# Autodesk Inventor assembly: Butterfly Drive Module_MIR1
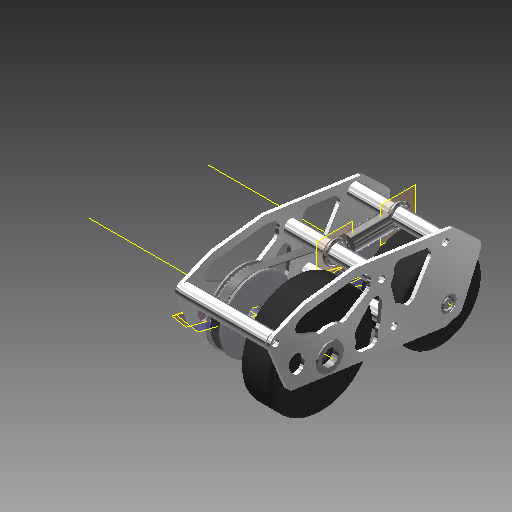
[picture p0: Inventor's stored thumbnail of the model, 512x512]
Saved by Autodesk Inventor 2019.4 (Build 234330000, 330)
## iProperties
Created: 2019-11-02
Part Number: Butterfly Drive Module_MIR1
Document SubType Name: Assembly
Designer: Mark
Mass: 2569.42 g
Surface Area: 2380.54 cm^2
Volume: 1171.75 cm^3
Density: 2.1928 g/cm^3
Author: admin
## Documents named in this file (12)
- C:\Users\admin\Desktop\FRC 2020 Engineering\GitHub\7738-CAD-prep\Butterfly Drive Mk2\Butterfly Module\Butterfly Drive Module_MIR1.iam
- C:\Users\admin\Desktop\FRC 2020 Engineering\GitHub\7738-CAD-prep\Butterfly Drive Mk2\Butterfly Module\100mm Mecanum StandIn_MIR1.ipt
- C:\Users\admin\Desktop\FRC 2020 Engineering\GitHub\7738-CAD-prep\Butterfly Drive Mk2\Butterfly Module\100mm Traction Wheel StandIn_MIR1.ipt
- C:\Users\admin\Desktop\FRC 2020 Engineering\GitHub\7738-CAD-prep\Butterfly Drive Mk2\Butterfly Module\Connector_MIR1.ipt
- C:\Users\admin\Desktop\FRC 2020 Engineering\GitHub\7738-CAD-prep\Butterfly Drive Mk2\Butterfly Module\F6802_MIR1.ipt
- C:\Users\admin\Desktop\FRC 2020 Engineering\GitHub\7738-CAD-prep\Butterfly Drive Mk2\Butterfly Module\M6GBTeye_MIR1.ipt
- C:\Users\admin\Desktop\FRC 2020 Engineering\GitHub\7738-CAD-prep\Butterfly Drive Mk2\Butterfly Module\Module Plate 1_MIR1.ipt
- C:\Users\admin\Desktop\FRC 2020 Engineering\GitHub\7738-CAD-prep\Butterfly Drive Mk2\Butterfly Module\Butterfly Drive Module\Design Accelerator\Synchronous Belts Transmission1_MIR1.iam
- C:\Users\admin\Desktop\FRC 2020 Engineering\GitHub\7738-CAD-prep\Butterfly Drive Mk2\Butterfly Module\Pneumatics Connector_MIR1.ipt
- C:\Users\admin\Desktop\FRC 2020 Engineering\GitHub\7738-CAD-prep\Butterfly Drive Mk2\Butterfly Module\F6004_MIR1.ipt
- C:\Users\admin\Desktop\FRC 2020 Engineering\GitHub\7738-CAD-prep\Butterfly Drive Mk2\Butterfly Module\Mecanum Axle_MIR1.ipt
- C:\Users\admin\Desktop\FRC 2020 Engineering\GitHub\7738-CAD-prep\Butterfly Drive Mk2\Butterfly Module\Butterfly Drive Module\Design Accelerator\Key Connection1_MIR1.iam
## Components (18 placed, 11 different names)
1. 100mm Mecanum StandIn_MIR1:1 — Flush:1, Mate:2, Mate:19, Mate:43, Angle:1
2. 100mm Traction Wheel StandIn_MIR1:1 — Flush:1, Mate:1
3. Connector_MIR1:1 — Mate:6, Mate:5, Mate:10, Mate:44
4. F6802_MIR1:1 — Mate:4, Mate:3, Mate:13, Mate:24, Flush:4
5. M6GBTeye_MIR1:1 — Mate:9, Mate:11, Mate:33
6. Module Plate 1_MIR1:1 — Mate:1, Mate:6, Mate:5, Mate:4, Mate:3, Mate:2, Mate:8, Mate:7, Mate:12, Mate:20, Mate:37, Mate:35, Mate:39, Mate:38, Mate:41, Mate:40
7. Connector_MIR1:2 — Mate:9, Mate:8, Mate:7
8. M6GBTeye_MIR1:2 — Mate:11, Mate:10, Flush:3
9. Synchronous Belts Transmission1_MIR1:1 [sub-assembly] — Mate:24, Mate:20, Mate:19, Mate:29, Mate:28, Mate:31, Angle:1
10. F6802_MIR1:2 — Mate:42
11. Pneumatics Connector_MIR1:1 — Flush:3, Mate:33, Mate:49
12. F6004_MIR1:1 — Mate:37, Mate:35
13. Connector_MIR1:3 — Mate:39, Mate:38, Mate:46, Mate:45
14. Connector_MIR1:4 — Mate:41, Mate:40
15. Mecanum Axle_MIR1:1 — Mate:43, Flush:4, Mate:42
16. Key Connection1_MIR1:1 [sub-assembly]
17. Module Plate 1_MIR1:2 — Mate:49, Mate:46, Mate:45, Mate:44, Mate:48, Mate:47
18. F6004_MIR1:2 — Mate:48, Mate:47
## Relationships (42: Mate 38, Flush 3, Angle 1)
- Flush:1: 100mm Mecanum StandIn_MIR1:1 ↔ 100mm Traction Wheel StandIn_MIR1:1
- Mate:1: 100mm Traction Wheel StandIn_MIR1:1 ↔ Module Plate 1_MIR1:1
- Mate:6 (0.3 mm): Connector_MIR1:1 ↔ Module Plate 1_MIR1:1
- Mate:5: Connector_MIR1:1 ↔ Module Plate 1_MIR1:1
- Mate:4 (0.3 mm): F6802_MIR1:1 ↔ Module Plate 1_MIR1:1
- Mate:3: F6802_MIR1:1 ↔ Module Plate 1_MIR1:1
- Mate:2: 100mm Mecanum StandIn_MIR1:1 ↔ Module Plate 1_MIR1:1
- Mate:9: M6GBTeye_MIR1:1 ↔ Connector_MIR1:2
- Mate:8 (0.3 mm): Module Plate 1_MIR1:1 ↔ Connector_MIR1:2
- Mate:7: Module Plate 1_MIR1:1 ↔ Connector_MIR1:2
- Mate:11: M6GBTeye_MIR1:1 ↔ M6GBTeye_MIR1:2
- Mate:10: Connector_MIR1:1 ↔ M6GBTeye_MIR1:2
- Mate:12: Module Plate 1_MIR1:1
- Mate:13: F6802_MIR1:1
- Mate:15
- Mate:14
- Mate:24: F6802_MIR1:1 ↔ Synchronous Belts Transmission1_MIR1:1
- Mate:20 (3 mm): Module Plate 1_MIR1:1 ↔ Synchronous Belts Transmission1_MIR1:1
- Mate:19 (3 mm): 100mm Mecanum StandIn_MIR1:1 ↔ Synchronous Belts Transmission1_MIR1:1
- Mate:29: Synchronous Belts Transmission1_MIR1:1
- Mate:28: Synchronous Belts Transmission1_MIR1:1
- Mate:32
- Mate:31: Synchronous Belts Transmission1_MIR1:1
- Mate:30
- Flush:3 (2 mm): M6GBTeye_MIR1:2 ↔ Pneumatics Connector_MIR1:1
- Mate:33: M6GBTeye_MIR1:1 ↔ Pneumatics Connector_MIR1:1
- Mate:37 (0.3 mm): Module Plate 1_MIR1:1 ↔ F6004_MIR1:1
- Mate:35: Module Plate 1_MIR1:1 ↔ F6004_MIR1:1
- Mate:39 (0.3 mm): Module Plate 1_MIR1:1 ↔ Connector_MIR1:3
- Mate:38: Module Plate 1_MIR1:1 ↔ Connector_MIR1:3
- Mate:41 (0.3 mm): Module Plate 1_MIR1:1 ↔ Connector_MIR1:4
- Mate:40: Module Plate 1_MIR1:1 ↔ Connector_MIR1:4
- Mate:43: 100mm Mecanum StandIn_MIR1:1 ↔ Mecanum Axle_MIR1:1
- Flush:4: F6802_MIR1:1 ↔ Mecanum Axle_MIR1:1
- Mate:42: F6802_MIR1:2 ↔ Mecanum Axle_MIR1:1
- Angle:1 (0 deg): 100mm Mecanum StandIn_MIR1:1 ↔ Synchronous Belts Transmission1_MIR1:1
- Mate:49 (52.5 mm): Pneumatics Connector_MIR1:1 ↔ Module Plate 1_MIR1:2
- Mate:46 (0.3 mm): Connector_MIR1:3 ↔ Module Plate 1_MIR1:2
- Mate:45: Connector_MIR1:3 ↔ Module Plate 1_MIR1:2
- Mate:44: Connector_MIR1:1 ↔ Module Plate 1_MIR1:2
- Mate:48 (0.3 mm): Module Plate 1_MIR1:2 ↔ F6004_MIR1:2
- Mate:47: Module Plate 1_MIR1:2 ↔ F6004_MIR1:2
